# Autodesk Inventor assembly: RFoF_Enclosure
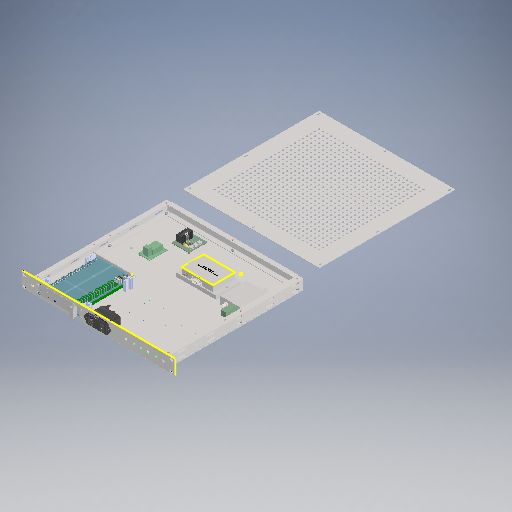
[picture p0: Inventor's stored thumbnail of the model, 512x512]
Saved by Autodesk Inventor 2025.3 (Build 293356000, 356)
## iProperties
Created: 2014-04-08
Part Number: RFoF_Enclosure
Document SubType Name: Assembly
Designer: alexanderpollak
Sending System: Autodesk Inventor 2012
Preprocessor: Autodesk Inventor 2012
Title: Z:\Eng\Products\Research and Development\PENDING TBC\GDI VD4001\VD4001-00-0117.stp
Author: DonFlagin
## Documents named in this file (23)
- C:\Users\sonata\Documents\SetiHCRO\Front-Page\Analog-Signal-Components\RFoF\1U-Enclosure\1PPS_10MHz_RX\RFoF_Enclosure.iam
- Sec_SecondStage_Enclosure.iam
- C:\Users\sonata\Documents\SetiHCRO\Front-Page\Analog-Signal-Components\RFoF\1U-Enclosure\1PPS_10MHz_RX\Parts\1UFrame\VC4084-00-0017.iam
- C:\Users\sonata\Documents\SetiHCRO\Front-Page\Analog-Signal-Components\RFoF\1U-Enclosure\1PPS_10MHz_RX\Parts\1UCaseTop.ipt
- C:\Users\sonata\Documents\SetiHCRO\Front-Page\Analog-Signal-Components\RFoF\1U-Enclosure\1PPS_10MHz_RX\Parts\HA2137-06-4009.ipt
- C:\Users\sonata\Documents\SetiHCRO\Front-Page\Analog-Signal-Components\RFoF\1U-Enclosure\1PPS_10MHz_RX\Parts\HA2112-06-5010.ipt
- C:\Users\sonata\Documents\SetiHCRO\Front-Page\Analog-Signal-Components\RFoF\1U-Enclosure\1PPS_10MHz_RX\Parts\HexNut_Schroff.ipt
- C:\Users\sonata\Documents\SetiHCRO\Front-Page\Analog-Signal-Components\RFoF\1U-Enclosure\1PPS_10MHz_RX\BottomPlate.ipt
- C:\Users\sonata\Documents\SetiHCRO\Front-Page\Analog-Signal-Components\RFoF\1U-Enclosure\1PPS_10MHz_RX\Parts\AC-Inlet\35718.iam
- C:\Users\sonata\Documents\SetiHCRO\Front-Page\Analog-Signal-Components\RFoF\1U-Enclosure\1PPS_10MHz_RX\Parts\Max-Power-6HP\13100151.iam
- C:\Users\sonata\Documents\SetiHCRO\Front-Page\Analog-Signal-Components\RFoF\1U-Enclosure\1PPS_10MHz_RX\SchroffThreadedInlay_30mm.ipt
- C:\Users\sonata\Documents\SetiHCRO\Front-Page\Analog-Signal-Components\RFoF\1U-Enclosure\1PPS_10MHz_RX\SchroffRailNoExtrusion_30mm_Left.ipt
- C:\Users\sonata\Documents\SetiHCRO\Front-Page\Analog-Signal-Components\RFoF\1U-Enclosure\1PPS_10MHz_RX\SchroffRailNoExtrusion_30mm_Right.ipt
- C:\Users\sonata\Documents\SetiHCRO\Front-Page\Analog-Signal-Components\RFoF\1U-Enclosure\1PPS_10MHz_RX\Parts\Hex_standoff_M2.5_5mm_noPole.ipt
- C:\Users\sonata\Documents\SetiHCRO\Front-Page\Analog-Signal-Components\RFoF\1U-Enclosure\1PPS_10MHz_RX\Parts\Voltage_Regulator_for_ZX60-14LN-S+\Voltage_Regulator_for_ZX60-14LN-S+.iam
- C:\Users\sonata\Documents\SetiHCRO\Front-Page\Analog-Signal-Components\RFoF\1U-Enclosure\1PPS_10MHz_RX\Parts\CaseScrew.ipt
- C:\Users\PaulLinke\Documents\Inventor\Content Center Files\R2025\en-US\AS 1427(07)\AS 1427 - M3 x 5(6) II.ipt
- C:\Users\PaulLinke\Documents\Inventor\Content Center Files\R2025\en-US\BS 4183(2)\BS 4183 - M2.5 x 4(1) I.ipt
- C:\Users\sonata\Documents\SetiHCRO\Front-Page\Analog-Signal-Components\RFoF\1U-Enclosure\1PPS_10MHz_RX\Parts\Schroff_Back_Stabilizer.ipt
- C:\Users\sonata\Documents\SetiHCRO\Front-Page\Analog-Signal-Components\RFoF\1U-Enclosure\1PPS_10MHz_RX\Parts\Splitter_PCB.ipt
- C:\Users\sonata\Documents\SetiHCRO\Front-Page\Analog-Signal-Components\RFoF\1U-Enclosure\1PPS_10MHz_RX\Parts\OZ600Receiver.iam
- C:\Users\sonata\Documents\SetiHCRO\Front-Page\Analog-Signal-Components\RFoF\1U-Enclosure\1PPS_10MHz_RX\FrontPanelFOStoTTL.ipt
- C:\Users\sonata\Documents\SetiHCRO\Front-Page\Analog-Signal-Components\RFoF\1U-Enclosure\1PPS_10MHz_RX\Parts\MeinbergReceiver.iam
## Components (55 placed, 22 different names)
1. 1UCaseFrame:1 [sub-assembly] — Mate:1, Mate:2, Flush:1, Flush:2, Mate:26, Mate:28, Mate:29, Mate:30, Mate:31, Mate:32, Mate:33, Mate:35, Mate:37, Mate:38, Mate:39, Mate:40, Mate:150, Flush:10
2. TopPlate:1 — Mate:1, Flush:2
3. CaseScrew:1 — Mate:33, Mate:40, Mate:41
4. CaseScrew:2 — Mate:31, Mate:38, Mate:43
5. CaseScrew:3 — Mate:32, Mate:39, Mate:42
6. CaseScrew:4 — Mate:30, Mate:37, Mate:44
7. CaseScrew:5 — Mate:26, Mate:27
8. CaseScrew:6 — Mate:29, Mate:35, Mate:36
9. CaseScrew:7 — Mate:28, Mate:34
10. FrontPanelScrew:1
11. FrontPanelScrew:2
12. FrontPanelNut:1
13. FrontPanelNut:2
14. BottomPlate:1 — Mate:2, Flush:1, Mate:8, Mate:12, Mate:16, Mate:20, Mate:27, Mate:34, Mate:36, Mate:41, Mate:42, Mate:43, Mate:44, Mate:75, Mate:96, Mate:97, Mate:100, Mate:101, Mate:102, Mate:103, Mate:104, Mate:105, Mate:106, Mate:107, Mate:108, Mate:109, Mate:110, Mate:111, Mate:132, Mate:133, Mate:134, Mate:141, Mate:149, Flush:10, Mate:151
15. ACInlet:1 [sub-assembly] — Mate:121, Mate:122
16. PSU:1 [sub-assembly] — Mate:22, Mate:23
17. SchroffThreadedInlay_25mm:1 — Mate:6, Mate:7, Mate:23
18. SchroffThreadedInlay_25mm:3 — Mate:18, Mate:19, Mate:22
19. SchroffRailNoExtrusion_30mm_Left:3 — Mate:18, Mate:19, Mate:20, Mate:24, Flush:8, Mate:98
20. SchroffRailNoExtrusion_30mm_Left:4 — Mate:12, Mate:25
21. SchroffRailNoExtrusion_30mm_Right:2 — Mate:16, Mate:24
22. SchroffRailNoExtrusion_30mm_Right:3 — Mate:6, Mate:7, Mate:8, Mate:25, Flush:9, Mate:99
23. Voltage_Regulator_for_ZX60-14LN-S+:2 [sub-assembly] — Mate:59, Mate:66, Mate:69, Mate:70
24. AS 1110 - Metric M2.5 x 6:13 — Mate:59
25. AS 1110 - Metric M2.5 x 6:17 — Mate:66
26. AS 1110 - Metric M2.5 x 6:19 — Mate:69
27. AS 1110 - Metric M2.5 x 6:21 — Mate:70, Mate:75
28. SchroffRailNoExtrusion_30mm_Right:4 — Mate:97, Flush:8, Mate:98, Mate:128, Mate:129
29. SchroffRailNoExtrusion_30mm_Left:5 — Mate:96, Flush:9, Mate:99, Mate:130, Mate:131
30. HA2137-06-4009:8 — Mate:101
31. HA2137-06-4009:9 — Mate:100
32. HA2137-06-4009:10 — Mate:111
33. HA2137-06-4009:11 — Mate:108
34. HA2137-06-4009:12 — Mate:109
35. HA2137-06-4009:13 — Mate:110
36. HA2137-06-4009:14 — Mate:107
37. HA2137-06-4009:15 — Mate:106
38. HA2137-06-4009:16 — Mate:104
39. HA2137-06-4009:17 — Mate:105
40. HA2137-06-4009:18 — Mate:103
41. HA2137-06-4009:19 — Mate:102
42. CaseScrew:1 — Mate:132
43. AS 1427 Z - Metric M3 x 5:1 — Mate:121
44. AS 1427 Z - Metric M3 x 5:2 — Mate:122
45. BS 4183 Cross Recessed Flat Countersunk Head Machine Screw - Metric M2.5 x 4:1
46. BS 4183 Cross Recessed Flat Countersunk Head Machine Screw - Metric M2.5 x 4:2
47. BS 4183 Cross Recessed Flat Countersunk Head Machine Screw - Metric M2.5 x 4:3
48. BS 4183 Cross Recessed Flat Countersunk Head Machine Screw - Metric M2.5 x 4:4
49. SchroffThreadedInlay_30mm:4 — Mate:130, Mate:131, Insert:3
50. SchroffThreadedInlay_30mm:5 — Mate:128, Mate:129, Insert:2
51. Schroff_Back_Stabilizer:1 — Insert:2, Insert:3
52. Splitter_PCB:1 — Mate:133, Mate:134
53. OZ600Receiver:2 [sub-assembly] — Mate:141, Mate:149
54. FrontPanelFOStoTTL:1 — Mate:150
55. MeinbergReceiver:1 [sub-assembly] — Mate:151
## Relationships (74: Mate 67, Flush 5, Insert 2)
- Mate:1: 1UCaseFrame:1 ↔ TopPlate:1
- Mate:2: 1UCaseFrame:1 ↔ BottomPlate:1
- Flush:1 (-0.762 mm): 1UCaseFrame:1 ↔ BottomPlate:1
- Flush:2 (0.762 mm): 1UCaseFrame:1 ↔ TopPlate:1
- Mate:6: SchroffThreadedInlay_25mm:1 ↔ SchroffRailNoExtrusion_30mm_Right:3
- Mate:7 (0.125 mm): SchroffThreadedInlay_25mm:1 ↔ SchroffRailNoExtrusion_30mm_Right:3
- Mate:8: BottomPlate:1 ↔ SchroffRailNoExtrusion_30mm_Right:3
- Mate:12: BottomPlate:1 ↔ SchroffRailNoExtrusion_30mm_Left:4
- Mate:16: BottomPlate:1 ↔ SchroffRailNoExtrusion_30mm_Right:2
- Mate:18: SchroffThreadedInlay_25mm:3 ↔ SchroffRailNoExtrusion_30mm_Left:3
- Mate:19 (0.125 mm): SchroffThreadedInlay_25mm:3 ↔ SchroffRailNoExtrusion_30mm_Left:3
- Mate:20: BottomPlate:1 ↔ SchroffRailNoExtrusion_30mm_Left:3
- Mate:22: PSU:1 ↔ SchroffThreadedInlay_25mm:3
- Mate:23: PSU:1 ↔ SchroffThreadedInlay_25mm:1
- Mate:24: SchroffRailNoExtrusion_30mm_Left:3 ↔ SchroffRailNoExtrusion_30mm_Right:2
- Mate:25: SchroffRailNoExtrusion_30mm_Left:4 ↔ SchroffRailNoExtrusion_30mm_Right:3
- Mate:26: 1UCaseFrame:1 ↔ CaseScrew:5
- Mate:27: CaseScrew:5 ↔ BottomPlate:1
- Mate:28: 1UCaseFrame:1 ↔ CaseScrew:7
- Mate:29: 1UCaseFrame:1 ↔ CaseScrew:6
- Mate:30: 1UCaseFrame:1 ↔ CaseScrew:4
- Mate:31: 1UCaseFrame:1 ↔ CaseScrew:2
- Mate:32: 1UCaseFrame:1 ↔ CaseScrew:3
- Mate:33: 1UCaseFrame:1 ↔ CaseScrew:1
- Mate:34: CaseScrew:7 ↔ BottomPlate:1
- Mate:35: 1UCaseFrame:1 ↔ CaseScrew:6
- Mate:36: CaseScrew:6 ↔ BottomPlate:1
- Mate:37: 1UCaseFrame:1 ↔ CaseScrew:4
- Mate:38: 1UCaseFrame:1 ↔ CaseScrew:2
- Mate:39: 1UCaseFrame:1 ↔ CaseScrew:3
- Mate:40: 1UCaseFrame:1 ↔ CaseScrew:1
- Mate:41: CaseScrew:1 ↔ BottomPlate:1
- Mate:42: CaseScrew:3 ↔ BottomPlate:1
- Mate:43: CaseScrew:2 ↔ BottomPlate:1
- Mate:44: CaseScrew:4 ↔ BottomPlate:1
- Mate:59: Voltage_Regulator_for_ZX60-14LN-S+:2 ↔ AS 1110 - Metric M2.5 x 6:13
- Mate:66: Voltage_Regulator_for_ZX60-14LN-S+:2 ↔ AS 1110 - Metric M2.5 x 6:17
- Mate:69: Voltage_Regulator_for_ZX60-14LN-S+:2 ↔ AS 1110 - Metric M2.5 x 6:19
- Mate:70: Voltage_Regulator_for_ZX60-14LN-S+:2 ↔ AS 1110 - Metric M2.5 x 6:21
- Mate:75: BottomPlate:1 ↔ AS 1110 - Metric M2.5 x 6:21
- Mate:96: BottomPlate:1 ↔ SchroffRailNoExtrusion_30mm_Left:5
- Mate:97: BottomPlate:1 ↔ SchroffRailNoExtrusion_30mm_Right:4
- Flush:8: SchroffRailNoExtrusion_30mm_Left:3 ↔ SchroffRailNoExtrusion_30mm_Right:4
- Flush:9: SchroffRailNoExtrusion_30mm_Right:3 ↔ SchroffRailNoExtrusion_30mm_Left:5
- Mate:98 (114 mm): SchroffRailNoExtrusion_30mm_Left:3 ↔ SchroffRailNoExtrusion_30mm_Right:4
- Mate:99 (114 mm): SchroffRailNoExtrusion_30mm_Right:3 ↔ SchroffRailNoExtrusion_30mm_Left:5
- Mate:100: BottomPlate:1 ↔ HA2137-06-4009:9
- Mate:101: BottomPlate:1 ↔ HA2137-06-4009:8
- Mate:102: BottomPlate:1 ↔ HA2137-06-4009:19
- Mate:103: BottomPlate:1 ↔ HA2137-06-4009:18
- Mate:104: BottomPlate:1 ↔ HA2137-06-4009:16
- Mate:105: BottomPlate:1 ↔ HA2137-06-4009:17
- Mate:106: BottomPlate:1 ↔ HA2137-06-4009:15
- Mate:107: BottomPlate:1 ↔ HA2137-06-4009:14
- Mate:108: BottomPlate:1 ↔ HA2137-06-4009:11
- Mate:109: BottomPlate:1 ↔ HA2137-06-4009:12
- Mate:110: BottomPlate:1 ↔ HA2137-06-4009:13
- Mate:111: BottomPlate:1 ↔ HA2137-06-4009:10
- Mate:121: ACInlet:1 ↔ AS 1427 Z - Metric M3 x 5:1
- Mate:122: ACInlet:1 ↔ AS 1427 Z - Metric M3 x 5:2
- Mate:128 (0.125 mm): SchroffRailNoExtrusion_30mm_Right:4 ↔ SchroffThreadedInlay_30mm:5
- Mate:129: SchroffRailNoExtrusion_30mm_Right:4 ↔ SchroffThreadedInlay_30mm:5
- Mate:130: SchroffRailNoExtrusion_30mm_Left:5 ↔ SchroffThreadedInlay_30mm:4
- Mate:131 (0.125 mm): SchroffRailNoExtrusion_30mm_Left:5 ↔ SchroffThreadedInlay_30mm:4
- Insert:2 (2.2 mm): SchroffThreadedInlay_30mm:5 ↔ Schroff_Back_Stabilizer:1
- Insert:3 (2.2 mm): SchroffThreadedInlay_30mm:4 ↔ Schroff_Back_Stabilizer:1
- Mate:132: BottomPlate:1 ↔ CaseScrew:1
- Mate:133 (4 mm): BottomPlate:1 ↔ Splitter_PCB:1
- Mate:134: BottomPlate:1 ↔ Splitter_PCB:1
- Mate:141: BottomPlate:1 ↔ OZ600Receiver:2
- Mate:149: BottomPlate:1 ↔ OZ600Receiver:2
- Mate:150: 1UCaseFrame:1 ↔ FrontPanelFOStoTTL:1
- Flush:10: 1UCaseFrame:1 ↔ BottomPlate:1
- Mate:151: BottomPlate:1 ↔ MeinbergReceiver:1
